# Autodesk Inventor assembly: SP40-10 MARCO HOJA CORREDERA 1131x695
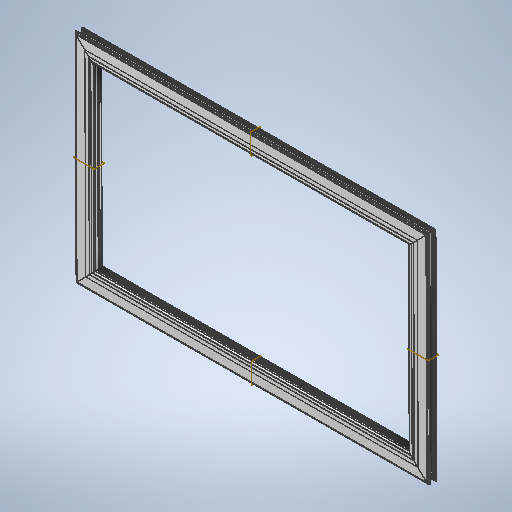
[picture p0: Inventor's stored thumbnail of the model, 512x512]
Saved by Autodesk Inventor 2025 (Build 290162000, 162)
## iProperties
Created: 2026-02-17
Part Number: SP40-10 MARCO HOJA CORREDERA 1131x695
Document SubType Name: Assembly
Designer: Frank
Author: Frank
## Documents named in this file (5)
- C:\Users\Frank\OneDrive\CARPINTERIA ALUMINIO\PUERTAS Y VENTANAS\VENTANAS\VENTANAS\PIEZAS\SP40-10 MARCO HOJA CORREDERA 1131x695.iam
- C:\Users\Frank\OneDrive\CARPINTERIA ALUMINIO\PUERTAS Y VENTANAS\VENTANAS\VENTANAS\PIEZAS\SP40-10 HOJA CORREDERA 1131 mm.ipt
- C:\Users\Frank\OneDrive\CARPINTERIA ALUMINIO\PUERTAS Y VENTANAS\VENTANAS\VENTANAS\PIEZAS\SP40-10 HOJA CORREDERA 695 mm.ipt
- C:\Users\Frank\OneDrive\CARPINTERIA ALUMINIO\PUERTAS Y VENTANAS\VENTANAS\VENTANAS\PIEZAS\SP40-10 HOJA CORREDERA 695 mm_MIR.ipt
- C:\Users\Frank\OneDrive\CARPINTERIA ALUMINIO\PUERTAS Y VENTANAS\VENTANAS\VENTANAS\PIEZAS\SP40-10 HOJA CORREDERA 1131 mm_MIR.ipt
## Components (4 placed, 4 different names)
1. SP40-10 HOJA CORREDERA 1131 mm:1 — Coincidencia:1, Coincidencia:2, Coincidencia:3, Coincidencia:4, Coincidencia:5, Coincidencia:6, Coincidencia:7, Coincidencia:8
2. SP40-10 HOJA CORREDERA 695 mm:1 — Coincidencia:3, Coincidencia:4, Coincidencia:5
3. SP40-10 HOJA CORREDERA 695 mm_MIR:1 — Coincidencia:6, Coincidencia:7, Coincidencia:8
4. SP40-10 HOJA CORREDERA 1131 mm_MIR:1 — Coincidencia:9, Coincidencia:10
## Relationships (10: Mate 10)
- Coincidencia:1 [Mate]: SP40-10 HOJA CORREDERA 1131 mm:1
- Coincidencia:2 [Mate]: SP40-10 HOJA CORREDERA 1131 mm:1
- Coincidencia:3 [Mate]: SP40-10 HOJA CORREDERA 1131 mm:1 ↔ SP40-10 HOJA CORREDERA 695 mm:1
- Coincidencia:4 [Mate]: SP40-10 HOJA CORREDERA 1131 mm:1 ↔ SP40-10 HOJA CORREDERA 695 mm:1
- Coincidencia:5 [Mate]: SP40-10 HOJA CORREDERA 1131 mm:1 ↔ SP40-10 HOJA CORREDERA 695 mm:1
- Coincidencia:6 [Mate]: SP40-10 HOJA CORREDERA 1131 mm:1 ↔ SP40-10 HOJA CORREDERA 695 mm_MIR:1
- Coincidencia:7 [Mate]: SP40-10 HOJA CORREDERA 1131 mm:1 ↔ SP40-10 HOJA CORREDERA 695 mm_MIR:1
- Coincidencia:8 [Mate]: SP40-10 HOJA CORREDERA 1131 mm:1 ↔ SP40-10 HOJA CORREDERA 695 mm_MIR:1
- Coincidencia:9 [Mate]: SP40-10 HOJA CORREDERA 1131 mm_MIR:1
- Coincidencia:10 [Mate]: SP40-10 HOJA CORREDERA 1131 mm_MIR:1
